# Autodesk Inventor assembly: HbIndexFingerForChild
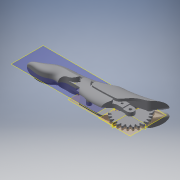
[picture p0: Inventor's stored thumbnail of the model, 180x180]
Saved by Autodesk Inventor 2017 (Build 210142000, 142)
## iProperties
Part Number: HbIndexFingerForChild
Material: 一般
Document SubType Name: Assembly
Designer: sktom
Author: sktom
## Documents named in this file (7)
- D:\OneDrive\CAD\hackberry\HACKberry-hardware\3D_69%\Hand\IndexFinger\HbIndexFingerForChild.iam
- D:\OneDrive\CAD\hackberry\HACKberry-hardware\3D_69%\Hand\IndexFinger\HbIndexInputLink02ForChild.ipt
- D:\OneDrive\CAD\hackberry\HACKberry-hardware\3D_69%\Hand\IndexFinger\HbIndexMiddle-DistalPhalanx02ForChild.ipt
- D:\OneDrive\CAD\hackberry\HACKberry-hardware\3D_69%\Hand\IndexFinger\HbIndexCouplerLink02ForChild.ipt
- D:\OneDrive\CAD\hackberry\HACKberry-hardware\3D_69%\Hand\IndexFinger\HbIndexCouplerLinkCover02ForChild.ipt
- D:\OneDrive\CAD\hackberry\HACKberry-hardware\3D_69%\Hand\IndexFinger\HbIndexProximalPhalanx03ForChild.ipt
- D:\OneDrive\CAD\hackberry\HACKberry-hardware\3D_69%\Hand\IndexFinger\HbIndexProximalPhalanxCover02ForChild.ipt
## Components (6 placed, 6 different names)
1. HbIndexInputLink02ForChild:1 — 挿入:4, 円柱状:1
2. HbIndexMiddle-DistalPhalanx02ForChild:1 — 挿入:1, 挿入:5
3. HbIndexCouplerLink02ForChild:1 — 挿入:1, 挿入:2, 挿入:3, 挿入:4
4. HbIndexCouplerLinkCover02ForChild:1 — 挿入:2, 挿入:3
5. HbIndexProximalPhalanx03ForChild:1 — 挿入:6, 挿入:7
6. HbIndexProximalPhalanxCover02ForChild:1 — 挿入:5, 挿入:6, 挿入:7, 円柱状:1
## Relationships (8: Insert 7, CylindricalJoint 1)
- 挿入:1 [Insert] (0.4 mm): HbIndexMiddle-DistalPhalanx02ForChild:1 ↔ HbIndexCouplerLink02ForChild:1
- 挿入:2 [Insert]: HbIndexCouplerLink02ForChild:1 ↔ HbIndexCouplerLinkCover02ForChild:1
- 挿入:3 [Insert]: HbIndexCouplerLink02ForChild:1 ↔ HbIndexCouplerLinkCover02ForChild:1
- 挿入:4 [Insert] (0.25 mm): HbIndexInputLink02ForChild:1 ↔ HbIndexCouplerLink02ForChild:1
- 挿入:5 [Insert] (0.4 mm): HbIndexMiddle-DistalPhalanx02ForChild:1 ↔ HbIndexProximalPhalanxCover02ForChild:1
- 挿入:6 [Insert]: HbIndexProximalPhalanx03ForChild:1 ↔ HbIndexProximalPhalanxCover02ForChild:1
- 挿入:7 [Insert]: HbIndexProximalPhalanx03ForChild:1 ↔ HbIndexProximalPhalanxCover02ForChild:1
- 円柱状:1 [CylindricalJoint]: HbIndexInputLink02ForChild:1 ↔ HbIndexProximalPhalanxCover02ForChild:1
